# Autodesk Inventor assembly: Loop Assembly
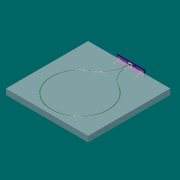
[picture p0: Inventor's stored thumbnail of the model, 180x180]
Saved by Autodesk Inventor 2016 (Build 200138000, 138)
## iProperties
Created: 2015-08-17
Part Number: Loop Assembly
Document SubType Name: Assembly
Designer: Cosmic
Author: Cosmic
## Documents named in this file (8)
- C:\Users\Sawaiz\Documents\3D\Inventor\SiPm ScintillatorTest Kit\Loop Assembly.iam
- C:\Users\Sawaiz\Documents\3D\Inventor\SiPm ScintillatorTest Kit\Scintillator Tile Loop.ipt
- C:\Users\Sawaiz\Documents\3D\Inventor\SiPm ScintillatorTest Kit\Fiber Loop.ipt
- C:\Users\Sawaiz\Documents\3D\Inventor\SiPm ScintillatorTest Kit\M3 Washer 95225A315.ipt
- C:\Users\Sawaiz\Documents\3D\Inventor\SiPm ScintillatorTest Kit\2mm spacer 93657A201.ipt
- C:\Users\Sawaiz\Documents\3D\Inventor\MPPC Sensor Board\MPPC Sensor V4 Populated.iam
- C:\Users\Sawaiz\Documents\3D\Inventor\Content Center Files\R2016\en-US\ANSI B18.6.7M(00)\ANSI B18.6.7M - M3x0.5 x 8(4).ipt
- C:\Users\Sawaiz\Documents\3D\Inventor\SiPm ScintillatorTest Kit\Scintillator.xlsx
## Components (9 placed, 6 different names)
1. Scintillator Tile Loop:1 — Flush:1, Tangent:1, Tangent:2, Tangent:3, Flush:2, Mate:12, Mate:13, Mate:14
2. Fiber Loop:1 — Flush:1, Tangent:1, Tangent:2, Tangent:3, Flush:2
3. M3 Washer 95225A315:1 — Mate:1, Mate:2, Mate:5
4. M3 Washer 95225A315:2 — Mate:3, Mate:4, Mate:6
5. 2mm spacer 93657A201:1 — Mate:1, Mate:2, Mate:8, Mate:10, Mate:14
6. 2mm spacer 93657A201:2 — Mate:3, Mate:4, Mate:7, Mate:11
7. MPPC Sensor V4 Populated:1 [sub-assembly] — Mate:5, Mate:6, Mate:7, Mate:8, Mate:9
8. Cross Recessed Pan Head Machine Screw - Type I - Metric M3x0.5 x 8:1 — Flush:3, Mate:9, Mate:10, Mate:12
9. Cross Recessed Pan Head Machine Screw - Type I - Metric M3x0.5 x 8:2 — Flush:3, Mate:11, Mate:13
## Relationships (20: Mate 14, Flush 3, Tangent 3)
- Flush:1: Scintillator Tile Loop:1 ↔ Fiber Loop:1
- Tangent:1 (0.15 mm): Scintillator Tile Loop:1 ↔ Fiber Loop:1
- Tangent:2 (0.15 mm): Scintillator Tile Loop:1 ↔ Fiber Loop:1
- Tangent:3 (0.15 mm): Scintillator Tile Loop:1 ↔ Fiber Loop:1
- Flush:2: Scintillator Tile Loop:1 ↔ Fiber Loop:1
- Mate:1: M3 Washer 95225A315:1 ↔ 2mm spacer 93657A201:1
- Mate:2: M3 Washer 95225A315:1 ↔ 2mm spacer 93657A201:1
- Mate:3: M3 Washer 95225A315:2 ↔ 2mm spacer 93657A201:2
- Mate:4: M3 Washer 95225A315:2 ↔ 2mm spacer 93657A201:2
- Mate:5: M3 Washer 95225A315:1 ↔ MPPC Sensor V4 Populated:1
- Mate:6: M3 Washer 95225A315:2 ↔ MPPC Sensor V4 Populated:1
- Mate:7: 2mm spacer 93657A201:2 ↔ MPPC Sensor V4 Populated:1
- Mate:8: 2mm spacer 93657A201:1 ↔ MPPC Sensor V4 Populated:1
- Flush:3: Cross Recessed Pan Head Machine Screw - Type I - Metric M3x0.5 x 8:1 ↔ Cross Recessed Pan Head Machine Screw - Type I - Metric M3x0.5 x 8:2
- Mate:9: MPPC Sensor V4 Populated:1 ↔ Cross Recessed Pan Head Machine Screw - Type I - Metric M3x0.5 x 8:1
- Mate:10: 2mm spacer 93657A201:1 ↔ Cross Recessed Pan Head Machine Screw - Type I - Metric M3x0.5 x 8:1
- Mate:11: 2mm spacer 93657A201:2 ↔ Cross Recessed Pan Head Machine Screw - Type I - Metric M3x0.5 x 8:2
- Mate:12: Scintillator Tile Loop:1 ↔ Cross Recessed Pan Head Machine Screw - Type I - Metric M3x0.5 x 8:1
- Mate:13: Scintillator Tile Loop:1 ↔ Cross Recessed Pan Head Machine Screw - Type I - Metric M3x0.5 x 8:2
- Mate:14: Scintillator Tile Loop:1 ↔ 2mm spacer 93657A201:1
## Named parameters: OpticalFiberClearence = 0.15 mm, MPPCClearence = 0.075 mm, FiberSensorClerence = 0.5 mm, OpticalFiberDiameter = 1 mm, ScintillatorThickness = 10 mm, SmallTrackDiameter = 175 mm, LargeTrackRatio = 3, ScintillatorEdgeClearence = 3 mm, ScintillatorWidth = 145 mm, ScintillatorHeight = 145 mm, ShallowTrackDepth = 1.3 mm, MPPCSensorClearence = 1.45 mm, MPPCSensorOffsett = 2.105 mm, MPPCWidth = 5.9 mm, MPPCHeight = 6.55 mm, FiberEdgeOffsett = 5 mm, MPPCDepth = 0 mm, LongFiberAngle = 30 deg, ShortFiberAngle = 78 deg, LoopLargeTrackRatio = 1.1, LoopSmallTrackDiameter = 90 mm, MountingScrewDepth = 4 mm, MountingScrewOffsett = 20 mm
